# Autodesk Inventor assembly: wheelAssembly01
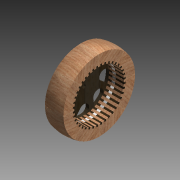
[picture p0: Inventor's stored thumbnail of the model, 180x180]
Saved by Autodesk Inventor 2013 (Build 170138000, 138)
## iProperties
Created: 2013-01-20
Part Number: wheelAssembly01
Document SubType Name: Assembly
Designer: Nano
Author: Nano
## Documents named in this file (3)
- C:\Users\Nano\Documents\InventorByron\InventorMasterProject\gyroPhone01\wheelAssembly01.iam
- C:\Users\Nano\Documents\InventorByron\InventorMasterProject\gyroPhone01\hubSpider.ipt
- C:\Users\Nano\Documents\InventorByron\InventorMasterProject\gyroPhone01\wedgeAssembly01.iam
## Components (9 placed, 2 different names)
1. hubSpider:1 — Mate:1, Insert:1
2. wedgeAssembly01:1 [sub-assembly]
3. wedgeAssembly01:2 [sub-assembly]
4. wedgeAssembly01:3 [sub-assembly]
5. wedgeAssembly01:4 [sub-assembly] — Insert:1
6. wedgeAssembly01:5 [sub-assembly]
7. wedgeAssembly01:6 [sub-assembly]
8. wedgeAssembly01:7 [sub-assembly] — Mate:1
9. wedgeAssembly01:8 [sub-assembly]
## Component patterns: (8 elements, first: wedgeAssembly01:1)
## Relationships (2: Mate 1, Insert 1)
- Mate:1: hubSpider:1 ↔ wedgeAssembly01:7
- Insert:1: hubSpider:1 ↔ wedgeAssembly01:4
